# Autodesk Inventor assembly: Lagerhalterung_ohne_Platte
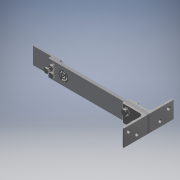
[picture p0: Inventor's stored thumbnail of the model, 180x180]
Saved by Autodesk Inventor 2018 (Build 220112000, 112)
## iProperties
Created: 2018-01-29
Part Number: Lagerhalterung_ohne_Platte
Material: Generisch
Document SubType Name: Assembly
Designer: Julian
Author: Julian
## Documents named in this file (12)
- C:\Users\Julian\Desktop\Schule\5AHME\Diplomarbeit\Git\fuettr_prototype\Mechanical\Inventorskizzen\Lagerhalterung_ohne_Platte.iam
- C:\Users\Julian\Desktop\Schule\5AHME\Diplomarbeit\Git\fuettr_prototype\Mechanical\Inventorskizzen\ISO 657-1 - L70x70x6-50.ipt
- C:\Users\Julian\Desktop\Schule\5AHME\Diplomarbeit\Git\fuettr_prototype\Mechanical\Inventorskizzen\Lagerstuetze.ipt
- C:\Users\Julian\Documents\Inventor\Content Center Files\R2018\de-DE\ISO 7090\ISO 7090 - 10 - 140 HV(1).ipt
- C:\Users\Julian\Documents\Inventor\Content Center Files\R2018\de-DE\ISO 7090\ISO 7090 - 8 - 140 HV(1).ipt
- C:\Users\Julian\Documents\Inventor\Content Center Files\R2018\de-DE\ISO 4017(1)\ISO 4017 - M10 x 35 - ISO.ipt
- C:\Users\Julian\Documents\Inventor\Content Center Files\R2018\de-DE\ISO 4032(2)\ISO 4032 - M10 - ISO.ipt
- C:\Users\Julian\Documents\Inventor\Content Center Files\R2018\de-DE\ISO 4032(2)\ISO 4032 - M8 - ISO.ipt
- C:\Users\Julian\Documents\Inventor\Content Center Files\R2018\de-DE\ISO 4017(1)\ISO 4017 - M8 x 25 - ISO.ipt
- C:\Users\Julian\Documents\Inventor\Content Center Files\R2018\de-DE\ISO 4017(1)\ISO 4017 - M8 x 40 - ISO.ipt
- C:\Users\Julian\Desktop\Schule\5AHME\Diplomarbeit\Git\fuettr_prototype\Mechanical\Inventorskizzen\Stuetzplatte.ipt
- C:\Users\Julian\Documents\Inventor\Content Center Files\R2018\de-DE\DIN 625 SKF(4)\DIN 625 SKF - SKF 6200-2Z.ipt
## Components (22 placed, 11 different names)
1. ISO 657-1 - L70x70x6-50:1 — Starr:1, Passend:1, Passend:2, Starr:3
2. ISO 657-1 - L70x70x6-50:2 — Starr:2, Starr:4, Starr:5
3. Lagerstuetze:1 — Starr:1, Starr:2, Drehbar:2, Fluchtend:1, Starr:9, Starr:10, Starr:18
4. ISO 7090 10 - 140 HV:1 — Passend:1, Passend:2, Starr:6
5. ISO 7090 10 - 140 HV:2 — Starr:3, Starr:7
6. ISO 7090 10 - 140 HV:3 — Starr:4, Starr:8
7. ISO 7090 10 - 140 HV:4 — Starr:5, Drehbar:1
8. ISO 7090 8 - 140 HV:1 — Starr:9, Starr:11
9. ISO 7090 8 - 140 HV:2 — Starr:13, Starr:15
10. ISO 7090 8 - 140 HV:3 — Starr:10, Starr:16
11. ISO 7090 8 - 140 HV:4 — Starr:12, Starr:14
12. ISO 4017 M10 x 35:1 — Starr:7
13. ISO 4017 M10 x 35:2 — Starr:6
14. ISO 4032 M10:1 — Starr:8
15. ISO 4032 M10:2 — Drehbar:1
16. ISO 4032 M8:1 — Starr:15, Starr:17
17. ISO 4032 M8:2 — Starr:14
18. ISO 4017 M8 x 25:1 — Starr:11
19. ISO 4017 M8 x 40:1 — Starr:17
20. ISO 4032 M8:3 — Starr:16
21. Stuetzplatte:1 — Drehbar:2, Fluchtend:1, Starr:12, Starr:13
22. DIN 625 SKF- beidseitig abgedeckt SKF 6200-2Z:1 — Starr:18
## Relationships (23: WeldJoint 18, Mate 2, RevoluteJoint 2, Flush 1)
- Starr:1 [WeldJoint]: ISO 657-1 - L70x70x6-50:1 ↔ Lagerstuetze:1
- Starr:2 [WeldJoint]: ISO 657-1 - L70x70x6-50:2 ↔ Lagerstuetze:1
- Passend:1 [Mate]: ISO 657-1 - L70x70x6-50:1 ↔ ISO 7090 10 - 140 HV:1
- Passend:2 [Mate]: ISO 657-1 - L70x70x6-50:1 ↔ ISO 7090 10 - 140 HV:1
- Starr:3 [WeldJoint]: ISO 657-1 - L70x70x6-50:1 ↔ ISO 7090 10 - 140 HV:2
- Starr:4 [WeldJoint]: ISO 657-1 - L70x70x6-50:2 ↔ ISO 7090 10 - 140 HV:3
- Starr:5 [WeldJoint]: ISO 657-1 - L70x70x6-50:2 ↔ ISO 7090 10 - 140 HV:4
- Starr:6 [WeldJoint]: ISO 7090 10 - 140 HV:1 ↔ ISO 4017 M10 x 35:2
- Starr:7 [WeldJoint]: ISO 7090 10 - 140 HV:2 ↔ ISO 4017 M10 x 35:1
- Starr:8 [WeldJoint]: ISO 7090 10 - 140 HV:3 ↔ ISO 4032 M10:1
- Drehbar:1 [RevoluteJoint]: ISO 7090 10 - 140 HV:4 ↔ ISO 4032 M10:2
- Drehbar:2 [RevoluteJoint]: Lagerstuetze:1 ↔ Stuetzplatte:1
- Fluchtend:1 [Flush]: Lagerstuetze:1 ↔ Stuetzplatte:1
- Starr:9 [WeldJoint]: Lagerstuetze:1 ↔ ISO 7090 8 - 140 HV:1
- Starr:10 [WeldJoint]: Lagerstuetze:1 ↔ ISO 7090 8 - 140 HV:3
- Starr:11 [WeldJoint]: ISO 7090 8 - 140 HV:1 ↔ ISO 4017 M8 x 25:1
- Starr:12 [WeldJoint]: ISO 7090 8 - 140 HV:4 ↔ Stuetzplatte:1
- Starr:13 [WeldJoint]: ISO 7090 8 - 140 HV:2 ↔ Stuetzplatte:1
- Starr:14 [WeldJoint]: ISO 7090 8 - 140 HV:4 ↔ ISO 4032 M8:2
- Starr:15 [WeldJoint]: ISO 7090 8 - 140 HV:2 ↔ ISO 4032 M8:1
- Starr:16 [WeldJoint]: ISO 7090 8 - 140 HV:3 ↔ ISO 4032 M8:3
- Starr:17 [WeldJoint]: ISO 4032 M8:1 ↔ ISO 4017 M8 x 40:1
- Starr:18 [WeldJoint]: Lagerstuetze:1 ↔ DIN 625 SKF- beidseitig abgedeckt SKF 6200-2Z:1
